# Autodesk Inventor assembly: тело фулл
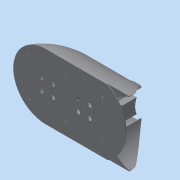
[picture p0: Inventor's stored thumbnail of the model, 180x180]
Saved by Autodesk Inventor 2019 (Build 230136000, 136)
## iProperties
Created: 2019-09-06
Part Number: тело фулл
Material: Типовые
Document SubType Name: Assembly
Designer: Iliga
Author: Iliga
## Documents named in this file (5)
- C:\Users\Максим\Desktop\САПР\Работы\ПД\робот\тело фулл.iam
- C:\Users\Максим\Desktop\САПР\Работы\ПД\робот\тело.ipt
- C:\Users\Максим\Desktop\САПР\Работы\ПД\робот\правое надкрылье.ipt
- C:\Users\Максим\Desktop\САПР\Работы\ПД\робот\рога.ipt
- C:\Users\Максим\Desktop\САПР\Работы\ПД\робот\хребет2.ipt
## Components (5 placed, 3 different names)
1. тело основа:1 — Заподлицо:3, Совмещение:2, Совмещение:3, Совмещение:8, Совмещение:9, Заподлицо:7, Совмещение:11
2. правое надкрылье:1 — Заподлицо:3, Совмещение:2, Совмещение:3, Совмещение:12
3. хребет2:4 — Совмещение:8, Заподлицо:5, Заподлицо:6, Совмещение:10, Заподлицо:7, Совмещение:13
4. хребет2:5 — Совмещение:9, Заподлицо:6, Совмещение:10
5. тело основа:2 — Совмещение:11, Совмещение:12, Совмещение:13
## Relationships (12: Mate 8, Flush 4)
- Заподлицо:3 [Flush]: тело основа:1 ↔ правое надкрылье:1
- Совмещение:2 [Mate]: тело основа:1 ↔ правое надкрылье:1
- Совмещение:3 [Mate]: тело основа:1 ↔ правое надкрылье:1
- Совмещение:8 [Mate]: тело основа:1 ↔ хребет2:4
- Заподлицо:5 [Flush]: хребет2:4
- Совмещение:9 [Mate]: тело основа:1 ↔ хребет2:5
- Заподлицо:6 [Flush]: хребет2:4 ↔ хребет2:5
- Совмещение:10 [Mate] (80 mm): хребет2:4 ↔ хребет2:5
- Заподлицо:7 [Flush]: тело основа:1 ↔ хребет2:4
- Совмещение:11 [Mate]: тело основа:1 ↔ тело основа:2
- Совмещение:12 [Mate]: правое надкрылье:1 ↔ тело основа:2
- Совмещение:13 [Mate] (15 mm): хребет2:4 ↔ тело основа:2
